# Autodesk Inventor assembly: ASY GBK длинная стенка
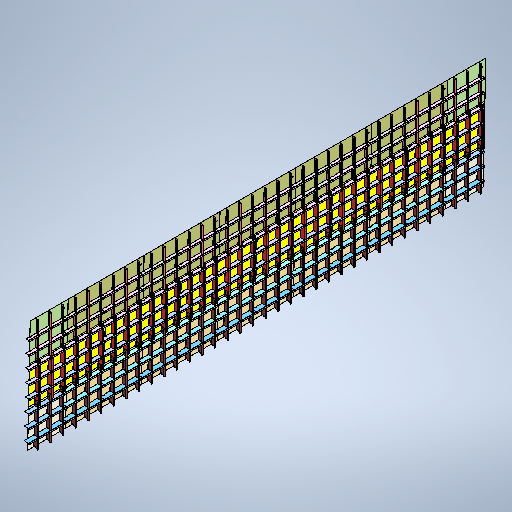
[picture p0: Inventor's stored thumbnail of the model, 512x512]
Saved by Autodesk Inventor 2026.2 (Build 302298010, 298A)
## iProperties
Created: 2026-05-20
Part Number: ASY GBK длинная стенка
Document SubType Name: Assembly
Designer: admin
Mass: 4.44159e+06 g
Surface Area: 2.86879e+06 cm^2
Volume: 565808 cm^3
Density: 7.85 g/cm^3
Author: admin
## Documents named in this file (6)
- C:\Users\admin\Documents\Inventor\GBK-Gubkinskiy\ASY GBK длинная стенка.iam
- C:\Users\admin\Documents\Inventor\GBK-Gubkinskiy\ASY GBK 1110 long wall shield 1.iam
- C:\Users\admin\Documents\Inventor\GBK-Gubkinskiy\ASY GBK 1120 long wall shield 2.iam
- C:\Users\admin\Documents\Inventor\GBK-Gubkinskiy\ASY GBK 1210 long wall shield 3.iam
- C:\Users\admin\Documents\Inventor\GBK-Gubkinskiy\ASY GBK 1310 long wall shield 4.iam
- C:\Users\admin\Documents\Inventor\GBK-Gubkinskiy\ASY GBK 1320 long wall shield 5.iam
## Components (20 placed, 5 different names)
1. ASY GBK 1110 long wall shield 1.iam:2 [sub-assembly] — Rigid:19
2. ASY GBK 1110 long wall shield 1.iam:1 [sub-assembly] — Flush:1, Mate:1, Mate:2, Rigid:14
3. ASY GBK 1120 long wall shield 2.iam:1 [sub-assembly] — Rigid:15, Rigid:16
4. ASY GBK 1210 long wall shield 3.iam:1 [sub-assembly]
5. ASY GBK 1310 long wall shield 4.iam:1 [sub-assembly] — Rigid:20
6. ASY GBK 1320 long wall shield 5.iam:1 [sub-assembly] — Rigid:20, Rigid:21
7. ASY GBK 1320 long wall shield 5.iam:2 [sub-assembly] — Rigid:21, Rigid:22
8. ASY GBK 1320 long wall shield 5.iam:3 [sub-assembly] — Rigid:22, Rigid:23
9. ASY GBK 1320 long wall shield 5.iam:4 [sub-assembly] — Rigid:23, Rigid:24
10. ASY GBK 1320 long wall shield 5.iam:5 [sub-assembly] — Rigid:24, Rigid:25
11. ASY GBK 1210 long wall shield 3.iam:2 [sub-assembly]
12. ASY GBK 1210 long wall shield 3.iam:3 [sub-assembly]
13. ASY GBK 1210 long wall shield 3.iam:4 [sub-assembly]
14. ASY GBK 1210 long wall shield 3.iam:5 [sub-assembly]
15. ASY GBK 1210 long wall shield 3.iam:6 [sub-assembly]
16. ASY GBK 1120 long wall shield 2.iam:2 [sub-assembly] — Rigid:14, Rigid:15
17. ASY GBK 1120 long wall shield 2.iam:3 [sub-assembly] — Rigid:16, Rigid:17
18. ASY GBK 1120 long wall shield 2.iam:4 [sub-assembly] — Rigid:17, Rigid:18
19. ASY GBK 1120 long wall shield 2.iam:5 [sub-assembly] — Rigid:18, Rigid:19
20. ASY GBK 1310 long wall shield 4.iam:2 [sub-assembly] — Rigid:25
## Relationships (22: WeldJoint 19, Mate 2, Flush 1)
- [WeldJoint]: ASY GBK 1110 long wall shield 1.iam:1 ↔ ASY GBK 1210 long wall shield 3.iam:1
- [WeldJoint]: ASY GBK 1210 long wall shield 3.iam:1 ↔ ASY GBK 1310 long wall shield 4.iam:1
- [WeldJoint] (1 mm): ASY GBK 1210 long wall shield 3.iam:1 ↔ ASY GBK 1210 long wall shield 3.iam:2
- [WeldJoint] (1 mm): ASY GBK 1210 long wall shield 3.iam:2 ↔ ASY GBK 1210 long wall shield 3.iam:3
- [WeldJoint] (1 mm): ASY GBK 1210 long wall shield 3.iam:3 ↔ ASY GBK 1210 long wall shield 3.iam:4
- [WeldJoint] (1 mm): ASY GBK 1210 long wall shield 3.iam:4 ↔ ASY GBK 1210 long wall shield 3.iam:5
- [WeldJoint] (1 mm): ASY GBK 1210 long wall shield 3.iam:5 ↔ ASY GBK 1210 long wall shield 3.iam:6
- Flush:1: ASY GBK 1110 long wall shield 1.iam:1
- Mate:1: ASY GBK 1110 long wall shield 1.iam:1
- Mate:2: ASY GBK 1110 long wall shield 1.iam:1
- Rigid:14 [WeldJoint] (1 mm): ASY GBK 1110 long wall shield 1.iam:1 ↔ ASY GBK 1120 long wall shield 2.iam:2
- Rigid:15 [WeldJoint] (1 mm): ASY GBK 1120 long wall shield 2.iam:1 ↔ ASY GBK 1120 long wall shield 2.iam:2
- Rigid:16 [WeldJoint] (1 mm): ASY GBK 1120 long wall shield 2.iam:1 ↔ ASY GBK 1120 long wall shield 2.iam:3
- Rigid:17 [WeldJoint] (1 mm): ASY GBK 1120 long wall shield 2.iam:3 ↔ ASY GBK 1120 long wall shield 2.iam:4
- Rigid:18 [WeldJoint] (1 mm): ASY GBK 1120 long wall shield 2.iam:4 ↔ ASY GBK 1120 long wall shield 2.iam:5
- Rigid:19 [WeldJoint] (1 mm): ASY GBK 1110 long wall shield 1.iam:2 ↔ ASY GBK 1120 long wall shield 2.iam:5
- Rigid:20 [WeldJoint] (1 mm): ASY GBK 1310 long wall shield 4.iam:1 ↔ ASY GBK 1320 long wall shield 5.iam:1
- Rigid:21 [WeldJoint] (1 mm): ASY GBK 1320 long wall shield 5.iam:1 ↔ ASY GBK 1320 long wall shield 5.iam:2
- Rigid:22 [WeldJoint] (1 mm): ASY GBK 1320 long wall shield 5.iam:2 ↔ ASY GBK 1320 long wall shield 5.iam:3
- Rigid:23 [WeldJoint] (1 mm): ASY GBK 1320 long wall shield 5.iam:3 ↔ ASY GBK 1320 long wall shield 5.iam:4
- Rigid:24 [WeldJoint] (1 mm): ASY GBK 1320 long wall shield 5.iam:4 ↔ ASY GBK 1320 long wall shield 5.iam:5
- Rigid:25 [WeldJoint] (1 mm): ASY GBK 1320 long wall shield 5.iam:5 ↔ ASY GBK 1310 long wall shield 4.iam:2
## Named parameters: Зазор_по_горизонту = 1 mm
